# Autodesk Inventor assembly: VersaWheel 2 sprockets center wheel for Drive in a Day 2013
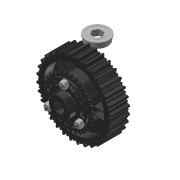
[picture p0: Inventor's stored thumbnail of the model, 180x180]
Saved by Autodesk Inventor 2013 (Build 170138000, 138)
## iProperties
Created: 2013-05-20
Part Number: VersaWheel 2 sprockets center wheel for Drive in a Day 2013
Document SubType Name: Assembly
Designer: Nemo
Author: Nemo
## Documents named in this file (7)
- H:\Nemo\Documents\Robotics\COTS Parts\Drive in a Day\VersaWheel 2 sprockets center wheel for Drive in a Day 2013.iam
- H:\Nemo\Documents\Robotics\Training Drive Base\Components\VexPro VersaWheel 4in.ipt
- H:\Nemo\Documents\Robotics\COTS Parts\Sprockets - VexPro #25\25 Sprocket 32T Vex.ipt
- H:\Nemo\Documents\Robotics\COTS Parts\Fasteners\8-32 locknut.ipt
- H:\Nemo\Documents\Robotics\COTS Parts\Fasteners\8-32 BHCS x2000.ipt
- H:\Nemo\Documents\Robotics\COTS Parts\Hubs\VersaHub 500 Hex.ipt
- H:\Nemo\Documents\Robotics\COTS Parts\Bearings - VexPro\Flanged Bearing - 0.5in Hex ID x 1.125in OD.ipt
## Components (11 placed, 6 different names)
1. VexPro VersaWheel 4in:1 — Insert:8
2. 25 Sprocket 32T Vex:1 — Insert:5, Mate:3
3. 25 Sprocket 32T Vex:2 — Insert:7
4. VersaHub 500 Hex:1 — Insert:5, Mate:3, Insert:6, Angle:1
5. Flanged Bearing - 0.5in Hex ID x 1.125in OD:1 — Insert:8, Angle:1
6. 8-32 locknut:1 — Insert:6
7. 8-32 BHCS x2000:1 — Insert:7
8. 8-32 locknut:2
9. 8-32 BHCS x2000:2
10. 8-32 locknut:3
11. 8-32 BHCS x2000:3
## Component patterns: (3 elements, first: 8-32 locknut:1 + 8-32 BHCS x2000:1)
## Relationships (10: Insert 6, Mate 3, Angle 1)
- [Insert]: VexPro VersaWheel 4in:1 ↔ 25 Sprocket 32T Vex:1
- [Mate]: VexPro VersaWheel 4in:1 ↔ 25 Sprocket 32T Vex:1
- [Insert]: VexPro VersaWheel 4in:1 ↔ 25 Sprocket 32T Vex:2
- [Mate]: VexPro VersaWheel 4in:1 ↔ 25 Sprocket 32T Vex:2
- Insert:5: 25 Sprocket 32T Vex:1 ↔ VersaHub 500 Hex:1
- Mate:3: 25 Sprocket 32T Vex:1 ↔ VersaHub 500 Hex:1
- Insert:6: VersaHub 500 Hex:1 ↔ 8-32 locknut:1
- Insert:7: 25 Sprocket 32T Vex:2 ↔ 8-32 BHCS x2000:1
- Insert:8: VexPro VersaWheel 4in:1 ↔ Flanged Bearing - 0.5in Hex ID x 1.125in OD:1
- Angle:1 (0 deg): VersaHub 500 Hex:1 ↔ Flanged Bearing - 0.5in Hex ID x 1.125in OD:1
